# Autodesk Inventor assembly: VelcroTrack1
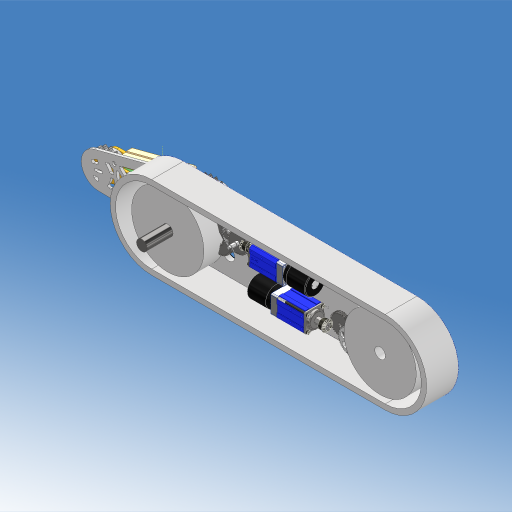
[picture p0: Inventor's stored thumbnail of the model, 512x512]
Saved by Autodesk Inventor 2024 (Build 280153000, 153)
## iProperties
Created: 2024-03-31
Part Number: VelcroTrack1
Document SubType Name: Assembly
Designer: seene
Author: seene
## Documents named in this file (11)
- C:\Users\seene\OneDrive\SBRT\Robocup Rescue\Drive\TestRigs\Other Ideas\VelcroTrack1.iam
- C:\Users\seene\OneDrive\SBRT\Robocup Rescue\Drive\TestRigs\MainDriveTestrig\Pulleys\BigPulley.ipt
- C:\Users\seene\OneDrive\SBRT\Robocup Rescue\Drive\MasterSketch - Copy.ipt
- C:\Users\seene\OneDrive\SBRT\Robocup Rescue\Drive\v1\FlipperMotorGearboxAssembly.iam
- C:\Users\seene\OneDrive\SBRT\Robocup Rescue\Drive\v1\TankFlipper.iam
- C:\Users\seene\OneDrive\SBRT\Robocup Rescue\Drive\v1\am-2460 35 Tooth CIM Gear.ipt
- C:\Users\seene\OneDrive\SBRT\Robocup Rescue\Drive\v1\Spur Gear (28 teeth).ipt
- C:\Users\seene\OneDrive\SBRT\Robocup Rescue\Drive\v1\am-2352 50 Tooth 20 DP 0.75 in. Hex Bore Steel Gear.ipt
- C:\Users\seene\OneDrive\SBRT\Robocup Rescue\Drive\v1\1439K211_1045 Carbon Steel Keyed Rotary Shaft.ipt
- C:\Users\seene\OneDrive\SBRT\Robocup Rescue\Drive\v1\am-0185 45 Tooth Gear 20 dp 500 Hex Bore.ipt
- C:\Users\seene\OneDrive\SBRT\Robocup Rescue\Drive\MasterSketch - Copy - Copy.ipt
## Components (17 placed, 10 different names)
1. BigPulley:1 — Mate:8, Flush:1, Mate:24, Mate:25
2. BigPulley:2 — Mate:9, Flush:1, Mate:23
3. MasterSketch - Copy:1 — Mate:2, Mate:3, Mate:4, Mate:5, Mate:6, Mate:7, Mate:8, Mate:9, Flush:2, Mate:10, Flush:3, Mate:11
4. FlipperMotorGearboxAssembly:1 [sub-assembly] — Mate:2, Mate:6, Mate:7
5. FlipperMotorGearboxAssembly:2 [sub-assembly] — Mate:3, Mate:4, Mate:5
6. MasterSketch - Copy:2 — Flush:2, Mate:10, Flush:3, Mate:12, Mate:14, Mate:15, Mate:17, Mate:18, Mate:19, Mate:20, Mate:22, Flush:12, Mate:25
7. TankFlipper:1 [sub-assembly] — Mate:11, Flush:6
8. am-2460 35 Tooth CIM Gear:1 — Mate:16
9. Spur Gear (28 teeth):1 — Mate:13, Flush:4, Flush:5, Mate:14, Flush:6
10. am-2352 50 Tooth 20 DP 0.75 in. Hex Bore Steel Gear:1 — Mate:12, Mate:13, Flush:4, Flush:5, Flush:7
11. 1439K211_1045 Carbon Steel Keyed Rotary Shaft:1 — Mate:15, Mate:16
12. am-0185 45 Tooth Gear 20 dp 500 Hex Bore:1 — Mate:17, Flush:7
13. am-0185 45 Tooth Gear 20 dp 500 Hex Bore:2 — Mate:18, Mate:19, Flush:10, Flush:11
14. am-2460 35 Tooth CIM Gear:2 — Mate:22, Flush:11
15. am-2352 50 Tooth 20 DP 0.75 in. Hex Bore Steel Gear:2 — Mate:20, Mate:21, Flush:8, Flush:9, Flush:10
16. Spur Gear (28 teeth):2 — Mate:21, Flush:8, Flush:9
17. MasterSketch - Copy - Copy:1 — Mate:23, Mate:24, Flush:12
## Relationships (36: Mate 24, Flush 12)
- Mate:2: MasterSketch - Copy:1 ↔ FlipperMotorGearboxAssembly:1
- Mate:3: MasterSketch - Copy:1 ↔ FlipperMotorGearboxAssembly:2
- Mate:4: MasterSketch - Copy:1 ↔ FlipperMotorGearboxAssembly:2
- Mate:5: MasterSketch - Copy:1 ↔ FlipperMotorGearboxAssembly:2
- Mate:6: MasterSketch - Copy:1 ↔ FlipperMotorGearboxAssembly:1
- Mate:7: MasterSketch - Copy:1 ↔ FlipperMotorGearboxAssembly:1
- Mate:8: BigPulley:1 ↔ MasterSketch - Copy:1
- Mate:9: BigPulley:2 ↔ MasterSketch - Copy:1
- Flush:1: BigPulley:1 ↔ BigPulley:2
- Flush:2: MasterSketch - Copy:1 ↔ MasterSketch - Copy:2
- Mate:10 (50.8 mm): MasterSketch - Copy:1 ↔ MasterSketch - Copy:2
- Flush:3: MasterSketch - Copy:1 ↔ MasterSketch - Copy:2
- Mate:11: MasterSketch - Copy:1 ↔ TankFlipper:1
- Mate:12: MasterSketch - Copy:2 ↔ am-2352 50 Tooth 20 DP 0.75 in. Hex Bore Steel Gear:1
- Mate:13 (17.145 mm): Spur Gear (28 teeth):1 ↔ am-2352 50 Tooth 20 DP 0.75 in. Hex Bore Steel Gear:1
- Flush:4: Spur Gear (28 teeth):1 ↔ am-2352 50 Tooth 20 DP 0.75 in. Hex Bore Steel Gear:1
- Flush:5: Spur Gear (28 teeth):1 ↔ am-2352 50 Tooth 20 DP 0.75 in. Hex Bore Steel Gear:1
- Mate:14 (1.5875 mm): MasterSketch - Copy:2 ↔ Spur Gear (28 teeth):1
- Flush:6: TankFlipper:1 ↔ Spur Gear (28 teeth):1
- Mate:15: MasterSketch - Copy:2 ↔ 1439K211_1045 Carbon Steel Keyed Rotary Shaft:1
- Mate:16: am-2460 35 Tooth CIM Gear:1 ↔ 1439K211_1045 Carbon Steel Keyed Rotary Shaft:1
- Mate:17: MasterSketch - Copy:2 ↔ am-0185 45 Tooth Gear 20 dp 500 Hex Bore:1
- Flush:7: am-2352 50 Tooth 20 DP 0.75 in. Hex Bore Steel Gear:1 ↔ am-0185 45 Tooth Gear 20 dp 500 Hex Bore:1
- Mate:18: MasterSketch - Copy:2 ↔ am-0185 45 Tooth Gear 20 dp 500 Hex Bore:2
- Mate:19: MasterSketch - Copy:2 ↔ am-0185 45 Tooth Gear 20 dp 500 Hex Bore:2
- Mate:20: MasterSketch - Copy:2 ↔ am-2352 50 Tooth 20 DP 0.75 in. Hex Bore Steel Gear:2
- Mate:21 (19.05 mm): am-2352 50 Tooth 20 DP 0.75 in. Hex Bore Steel Gear:2 ↔ Spur Gear (28 teeth):2
- Flush:8: am-2352 50 Tooth 20 DP 0.75 in. Hex Bore Steel Gear:2 ↔ Spur Gear (28 teeth):2
- Flush:9: am-2352 50 Tooth 20 DP 0.75 in. Hex Bore Steel Gear:2 ↔ Spur Gear (28 teeth):2
- Flush:10: am-0185 45 Tooth Gear 20 dp 500 Hex Bore:2 ↔ am-2352 50 Tooth 20 DP 0.75 in. Hex Bore Steel Gear:2
- Mate:22: MasterSketch - Copy:2 ↔ am-2460 35 Tooth CIM Gear:2
- Flush:11: am-0185 45 Tooth Gear 20 dp 500 Hex Bore:2 ↔ am-2460 35 Tooth CIM Gear:2
- Mate:23: BigPulley:2 ↔ MasterSketch - Copy - Copy:1
- Mate:24: BigPulley:1 ↔ MasterSketch - Copy - Copy:1
- Flush:12: MasterSketch - Copy:2 ↔ MasterSketch - Copy - Copy:1
- Mate:25 (0.4 mm): BigPulley:1 ↔ MasterSketch - Copy:2
